# Autodesk Inventor assembly: Main
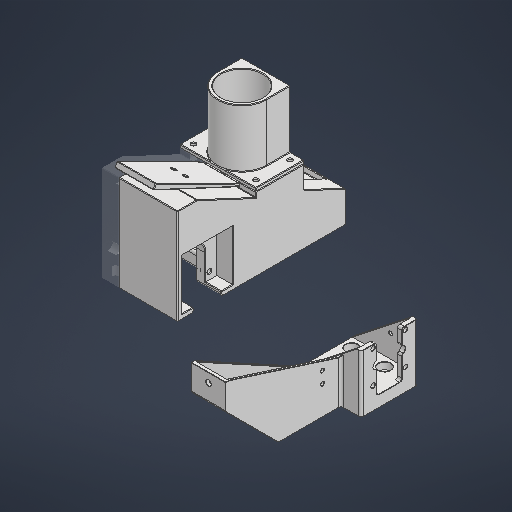
[picture p0: Inventor's stored thumbnail of the model, 512x512]
Saved by Autodesk Inventor 2025 (Build 290162010, 162A)
## iProperties
Created: 2025-10-23
Part Number: Main
Document SubType Name: Assembly
Designer: FizzyApple12
Author: FizzyApple12
## Documents named in this file (8)
- C:\Users\FizzyApple12\Desktop\connect4spill\mcad\Main.iam
- C:\Users\FizzyApple12\Desktop\connect4spill\mcad\Game-Piece.ipt
- C:\Users\FizzyApple12\Desktop\connect4spill\mcad\End-Effector\End-Effector.iam
- C:\Users\FizzyApple12\Desktop\connect4spill\mcad\Game-Piece-Funnel-Motor-Half.ipt
- C:\Users\FizzyApple12\Desktop\connect4spill\mcad\Game-Piece-Funnel-Enclosure-Half.ipt
- C:\Users\FizzyApple12\Desktop\connect4spill\mcad\Fabrication\Game-Piece-Funnel-Hopper.ipt
- C:\Users\FizzyApple12\Desktop\connect4spill\mcad\Fabrication\Game-Piece-Funnel-Pusher-Plate.ipt
- C:\Users\FizzyApple12\Desktop\connect4spill\mcad\Game-Piece-Funnel-Pusher-Carriage.ipt
## Components (7 placed, 7 different names)
1. Game-Piece:1
2. End-Effector:1 [sub-assembly]
3. Game-Piece-Funnel-Motor-Half:1 — Mate:1, Mate:2, Mate:3, Mate:4, Mate:5, Mate:7, Mate:8
4. Game-Piece-Funnel-Enclosure-Half:1 — Mate:1, Mate:2, Mate:3, Mate:6
5. Game-Piece-Funnel-Hopper:1 — Mate:4, Mate:5, Mate:6
6. Game-Piece-Funnel-Pusher-Plate:1 — Mate:7, Mate:8, Mate:9, Mate:10, Mate:11
7. Game-Piece-Funnel-Pusher-Carriage:1 — Mate:9, Mate:10, Mate:11
## Relationships (11: Mate 11)
- Mate:1: Game-Piece-Funnel-Motor-Half:1 ↔ Game-Piece-Funnel-Enclosure-Half:1
- Mate:2: Game-Piece-Funnel-Motor-Half:1 ↔ Game-Piece-Funnel-Enclosure-Half:1
- Mate:3: Game-Piece-Funnel-Motor-Half:1 ↔ Game-Piece-Funnel-Enclosure-Half:1
- Mate:4: Game-Piece-Funnel-Motor-Half:1 ↔ Game-Piece-Funnel-Hopper:1
- Mate:5: Game-Piece-Funnel-Motor-Half:1 ↔ Game-Piece-Funnel-Hopper:1
- Mate:6: Game-Piece-Funnel-Enclosure-Half:1 ↔ Game-Piece-Funnel-Hopper:1
- Mate:7: Game-Piece-Funnel-Motor-Half:1 ↔ Game-Piece-Funnel-Pusher-Plate:1
- Mate:8 (1 mm): Game-Piece-Funnel-Motor-Half:1 ↔ Game-Piece-Funnel-Pusher-Plate:1
- Mate:9: Game-Piece-Funnel-Pusher-Plate:1 ↔ Game-Piece-Funnel-Pusher-Carriage:1
- Mate:10: Game-Piece-Funnel-Pusher-Plate:1 ↔ Game-Piece-Funnel-Pusher-Carriage:1
- Mate:11: Game-Piece-Funnel-Pusher-Plate:1 ↔ Game-Piece-Funnel-Pusher-Carriage:1
